# Autodesk Inventor assembly: Asm1
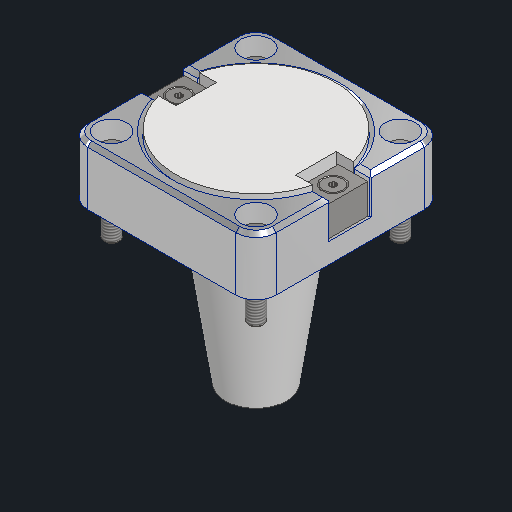
[picture p0: Inventor's stored thumbnail of the model, 512x512]
Saved by Autodesk Inventor 2024.3 (Build 283343000, 343)
## iProperties
Created: 2024-01-14
Part Number: Asm1
Document SubType Name: Assembly
Designer: fablabadmin
Author: fablabadmin
## Documents named in this file (6)
- C:\Users\fablabadmin\Documents\_Benjamin_S\_3dCAD\HHVerkstad\ToolHolder\TH1.iam
- C:\Users\fablabadmin\Documents\_Benjamin_S\_3dCAD\HHVerkstad\ToolHolder\SK40Collar.ipt
- C:\Users\fablabadmin\Documents\_Benjamin_S\_3dCAD\HHVerkstad\ToolHolder\TH1-001.ipt
- C:\Users\fablabadmin\Documents\_Benjamin_S\_3dCAD\HHVerkstad\ToolHolder\TH1-002.ipt
- C:\Users\fablabadmin\Documents\Inventor\Content Center Files\R2024\en-US\AS 1420\AS 1420 - 1973 - M6 x 25.ipt
- C:\Users\fablabadmin\Documents\Inventor\Content Center Files\R2024\en-US\ASME ANSI B18.3.5M(2)\ASME_ANSI B18.3.5M - M4x16(2).ipt
## Components (10 placed, 5 different names)
1. SK40Collar:1 — Flush:2
2. TH1-001:1 — Flush:1, Flush:2, Flush:3, Mate:1, Mate:2, Angle:1, Mate:3, Mate:4, Mate:5, Mate:6, Mate:7, Mate:8, Mate:9, Mate:10
3. TH1-002:1 — Flush:3, Mate:12
4. TH1-002:2 — Mate:1, Mate:2, Angle:1, Mate:11
5. AS 1420 - Metric M6 x 25:1 — Mate:5, Mate:10
6. AS 1420 - Metric M6 x 25:2 — Mate:6, Mate:9
7. AS 1420 - Metric M6 x 25:3 — Mate:3, Mate:7
8. AS 1420 - Metric M6 x 25:4 — Mate:4, Mate:8
9. Broached Hexagon Socket Flat Countersunk Head Cap Screws - Metric M4x16:1 — Mate:11
10. Broached Hexagon Socket Flat Countersunk Head Cap Screws - Metric M4x16:2 — Mate:12
## Relationships (16: Mate 12, Flush 3, Angle 1)
- Flush:1: TH1-001:1
- Flush:2: SK40Collar:1 ↔ TH1-001:1
- Flush:3: TH1-001:1 ↔ TH1-002:1
- Mate:1: TH1-001:1 ↔ TH1-002:2
- Mate:2: TH1-001:1 ↔ TH1-002:2
- Angle:1 (0 deg): TH1-001:1 ↔ TH1-002:2
- Mate:3: TH1-001:1 ↔ AS 1420 - Metric M6 x 25:3
- Mate:4: TH1-001:1 ↔ AS 1420 - Metric M6 x 25:4
- Mate:5: TH1-001:1 ↔ AS 1420 - Metric M6 x 25:1
- Mate:6: TH1-001:1 ↔ AS 1420 - Metric M6 x 25:2
- Mate:7: TH1-001:1 ↔ AS 1420 - Metric M6 x 25:3
- Mate:8: TH1-001:1 ↔ AS 1420 - Metric M6 x 25:4
- Mate:9: TH1-001:1 ↔ AS 1420 - Metric M6 x 25:2
- Mate:10: TH1-001:1 ↔ AS 1420 - Metric M6 x 25:1
- Mate:11: TH1-002:2 ↔ Broached Hexagon Socket Flat Countersunk Head Cap Screws - Metric M4x16:1
- Mate:12: TH1-002:1 ↔ Broached Hexagon Socket Flat Countersunk Head Cap Screws - Metric M4x16:2
